# Autodesk Inventor assembly: 01_pakutta_L
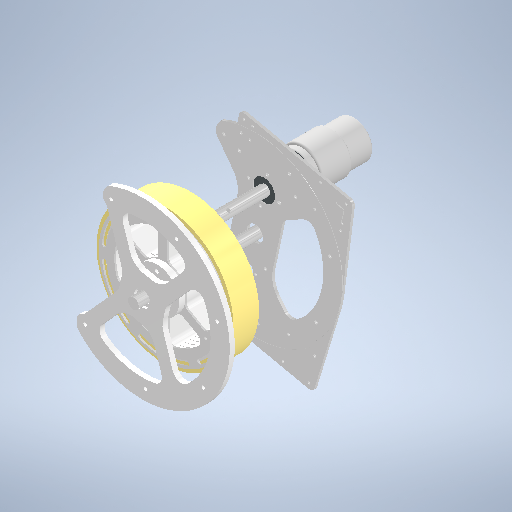
[picture p0: Inventor's stored thumbnail of the model, 512x512]
Saved by Autodesk Inventor 2025.1 (Build 291241000, 241)
## iProperties
Created: 2024-10-03
Part Number: 01_pakutta_L
Document SubType Name: Assembly
Designer: yuki0520
Author: yuki0520
## Documents named in this file (10)
- C:\Users\yuki0520\OneDrive\ドキュメント\Inventor\2025_nhk\tanaka\nageru\pakuriz\01_pakutta_L.iam
- C:\Users\yuki0520\OneDrive\ドキュメント\Inventor\2025_nhk\tanaka\nageru\pakuriz\tire.iam
- C:\Users\yuki0520\OneDrive\ドキュメント\Inventor\2025_nhk\tanaka\nageru\pakuriz\TH22_POM_handle_sn.ipt
- C:\Users\yuki0520\OneDrive\ドキュメント\Inventor\2025_nhk\tanaka\nageru\pakuriz\TH22_Bar_roller_sn.ipt
- C:\Users\yuki0520\OneDrive\ドキュメント\Inventor\2025_nhk\tanaka\inventorパーツリスト\モーター\775\RS-775GM.ipt
- C:\Users\yuki0520\OneDrive\ドキュメント\Inventor\2025_nhk\tanaka\inventorパーツリスト\モーター\775\RS-775GM_004GH_sn.ipt
- C:\Users\yuki0520\OneDrive\ドキュメント\Inventor\2025_nhk\tanaka\nageru\pakuriz\TH22_Bar_motor_roller_sn.ipt
- C:\Users\yuki0520\OneDrive\ドキュメント\Inventor\2025_nhk\tanaka\nageru\pakuriz\TH22_AlBoard_roller_775_L_sn.ipt
- C:\Users\yuki0520\OneDrive\ドキュメント\Inventor\2025_nhk\tanaka\nageru\pakuriz\poll_8_4_121.2.ipt
- C:\Users\yuki0520\OneDrive\ドキュメント\Inventor\2025_nhk\tanaka\nageru\pakuriz\TH22_3DP_cover_fixer_sn.ipt
## Components (9 placed, 9 different names)
1. tire:1 [sub-assembly] — メイト:1, メイト:3
2. TH22_POM_handle_sn:1 — メイト:2, 挿入:3, フラッシュ:1
3. TH22_Bar_roller_sn:1 — メイト:1, メイト:2, メイト:3, メイト:6, フラッシュ:1
4. RS-775GM:1 — メイト:4, 正接:1
5. RS-775GM_004GH_sn:1 — メイト:4, 正接:1, メイト:5, 挿入:1, 挿入:2, メイト:7
6. TH22_Bar_motor_roller_sn:1 — メイト:5, メイト:7
7. TH22_AlBoard_roller_775_L_sn:1 — 挿入:1, 挿入:2, メイト:6, 挿入:4
8. poll_8_4_121.2:1 — 挿入:3, 挿入:4, 挿入:5
9. TH22_3DP_cover_fixer_sn:1 — 挿入:5
## Relationships (14: Mate 7, Insert 5, Tangent 1, Flush 1)
- メイト:1 [Mate]: tire:1 ↔ TH22_Bar_roller_sn:1
- メイト:2 [Mate]: TH22_POM_handle_sn:1 ↔ TH22_Bar_roller_sn:1
- メイト:3 [Mate]: tire:1 ↔ TH22_Bar_roller_sn:1
- メイト:4 [Mate]: RS-775GM:1 ↔ RS-775GM_004GH_sn:1
- 正接:1 [Tangent]: RS-775GM:1 ↔ RS-775GM_004GH_sn:1
- メイト:5 [Mate]: RS-775GM_004GH_sn:1 ↔ TH22_Bar_motor_roller_sn:1
- 挿入:1 [Insert]: RS-775GM_004GH_sn:1 ↔ TH22_AlBoard_roller_775_L_sn:1
- 挿入:2 [Insert]: RS-775GM_004GH_sn:1 ↔ TH22_AlBoard_roller_775_L_sn:1
- メイト:6 [Mate]: TH22_Bar_roller_sn:1 ↔ TH22_AlBoard_roller_775_L_sn:1
- 挿入:3 [Insert]: TH22_POM_handle_sn:1 ↔ poll_8_4_121.2:1
- 挿入:4 [Insert]: TH22_AlBoard_roller_775_L_sn:1 ↔ poll_8_4_121.2:1
- メイト:7 [Mate]: RS-775GM_004GH_sn:1 ↔ TH22_Bar_motor_roller_sn:1
- フラッシュ:1 [Flush] (-10 mm): TH22_POM_handle_sn:1 ↔ TH22_Bar_roller_sn:1
- 挿入:5 [Insert]: poll_8_4_121.2:1 ↔ TH22_3DP_cover_fixer_sn:1
